# Autodesk Inventor assembly: IPT_TRACK_assembly
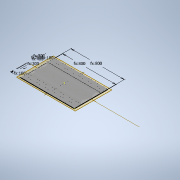
[picture p0: Inventor's stored thumbnail of the model, 180x180]
Saved by Autodesk Inventor 2021 (Build 250183000, 183)
## iProperties
Created: 2021-02-13
Part Number: IPT_TRACK_assembly
Document SubType Name: Assembly
Designer: phamv
Author: phamv
## Documents named in this file (3)
- C:\Users\phamv\OneDrive\UoA\2020 SUMMER\2020-srw-rc-car\CoilDesign\DEXTER_WORKSPACE\CAD stuff\Final_CAD\IPT_TRACK_assembly.iam
- C:\Users\phamv\OneDrive\UoA\2020 SUMMER\2020-srw-rc-car\CoilDesign\DEXTER_WORKSPACE\CAD stuff\Final_CAD\ferrite_layer_dex_1R1.ipt
- C:\Users\phamv\OneDrive\UoA\2020 SUMMER\2020-srw-rc-car\CoilDesign\DEXTER_WORKSPACE\CAD stuff\Final_CAD\primary_coil_0R2.ipt
## Components (2 placed, 2 different names)
1. ferrite_layer_dex_1R1:1 — Rigid:1
2. primary_coil_0R2:1 — Rigid:1
## Relationships (1: WeldJoint 1)
- Rigid:1 [WeldJoint]: ferrite_layer_dex_1R1:1 ↔ primary_coil_0R2:1
